# Autodesk Inventor assembly: Frame Assembly
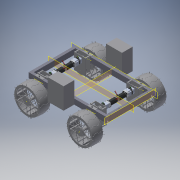
[picture p0: Inventor's stored thumbnail of the model, 180x180]
Saved by Autodesk Inventor 2019 (Build 230136000, 136)
## iProperties
Created: 2018-10-28
Part Number: Frame Assembly
Document SubType Name: Assembly
Designer: Swapnil
Author: Swapnil
## Documents named in this file (6)
- C:\Users\Alex Barnett\Documents\Machine Design\PR2\CAD\Frame\Frame Assembly.iam
- C:\Users\Alex Barnett\Documents\Machine Design\PR2\CAD\Frame\Resized frame.ipt
- C:\Users\Alex Barnett\Documents\Machine Design\PR2\CAD\Frame\Motor Mount.iam
- C:\Users\Alex Barnett\Documents\Machine Design\PR2\CAD\Frame\Full Wheel.iam
- C:\Users\Alex Barnett\Documents\Machine Design\PR2\CAD\Frame\Electrical Box Placeholder.ipt
- C:\Users\Alex Barnett\Documents\Machine Design\PR2\CAD\Frame\Electrical Box Placeholder_MIR.ipt
## Components (11 placed, 5 different names)
1. Resized frame:1 — Mate:1, Mate:2, Mate:3, Mate:4, Mate:5, Mate:6, Mate:7, Mate:8, Mate:14, Flush:5
2. Motor Mount:1 [sub-assembly] — Mate:1, Mate:2, Mate:12, Flush:4, Mate:13
3. Motor Mount:2 [sub-assembly] — Mate:3, Mate:4, Mate:10, Flush:2, Mate:13
4. Motor Mount:3 [sub-assembly] — Mate:5, Mate:6, Mate:11, Flush:3
5. Motor Mount:4 [sub-assembly] — Mate:7, Mate:8, Mate:9, Flush:1
6. Full Wheel:1 [sub-assembly] — Mate:10, Flush:2
7. Full Wheel:2 [sub-assembly] — Mate:9, Flush:1
8. Full Wheel:3 [sub-assembly] — Mate:11, Flush:3
9. Full Wheel:4 [sub-assembly] — Mate:12, Flush:4
10. Electrical Box Placeholder:1 — Mate:14, Flush:5
11. Electrical Box Placeholder_MIR:1
## Relationships (19: Mate 14, Flush 5)
- Mate:1: Resized frame:1 ↔ Motor Mount:1
- Mate:2: Resized frame:1 ↔ Motor Mount:1
- Mate:3: Resized frame:1 ↔ Motor Mount:2
- Mate:4: Resized frame:1 ↔ Motor Mount:2
- Mate:5: Resized frame:1 ↔ Motor Mount:3
- Mate:6: Resized frame:1 ↔ Motor Mount:3
- Mate:7: Resized frame:1 ↔ Motor Mount:4
- Mate:8: Resized frame:1 ↔ Motor Mount:4
- Mate:9: Motor Mount:4 ↔ Full Wheel:2
- Flush:1: Motor Mount:4 ↔ Full Wheel:2
- Mate:10: Motor Mount:2 ↔ Full Wheel:1
- Flush:2: Motor Mount:2 ↔ Full Wheel:1
- Mate:11: Motor Mount:3 ↔ Full Wheel:3
- Flush:3: Motor Mount:3 ↔ Full Wheel:3
- Mate:12: Motor Mount:1 ↔ Full Wheel:4
- Flush:4: Motor Mount:1 ↔ Full Wheel:4
- Mate:13: Motor Mount:1 ↔ Motor Mount:2
- Mate:14: Resized frame:1 ↔ Electrical Box Placeholder:1
- Flush:5: Resized frame:1 ↔ Electrical Box Placeholder:1
